# Autodesk Inventor assembly: McCrea_walle_drifter_walle
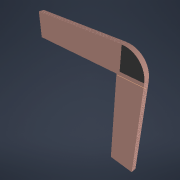
[picture p0: Inventor's stored thumbnail of the model, 180x180]
Saved by Autodesk Inventor 2022 (Build 260153000, 153)
## iProperties
Created: 2022-02-12
Part Number: McCrea_walle_drifter_walle
Document SubType Name: Assembly
Designer: MatusBarany
Author: MatusBarany
## Documents named in this file (4)
- C:\Users\MatusBarany\Documents\Inventor\wall-e\assembly\McCrea_walle_drifter_walle.iam
- C:\Users\MatusBarany\Documents\Inventor\wall-e\matus\plocha\McCrea_most_cesta_walle.ipt
- C:\Users\MatusBarany\Documents\Inventor\wall-e\matus\plocha\McCrea_zakruta_walle.ipt
- C:\Users\MatusBarany\Documents\Inventor\wall-e\assembly\McCrea_WALLE_bez_HEAD_walle.iam
## Components (6 placed, 3 different names)
1. McCrea_most_cesta_walle:1 — Mate:1, Flush:1, Mate:2, Mate:3, Flush:3, Mate:5, Mate:6
2. McCrea_zakruta_walle:1 — Mate:1, Flush:1, Mate:2, Mate:4, Flush:2
3. McCrea_WALLE_bez_HEAD_walle:1 [sub-assembly] — Mate:3
4. McCrea_most_cesta_walle:2 — Mate:4, Flush:2, Flush:3
5. McCrea_WALLE_bez_HEAD_walle:2 [sub-assembly] — Mate:5
6. McCrea_WALLE_bez_HEAD_walle:3 [sub-assembly] — Mate:6
## Relationships (9: Mate 6, Flush 3)
- Mate:1: McCrea_most_cesta_walle:1 ↔ McCrea_zakruta_walle:1
- Flush:1: McCrea_most_cesta_walle:1 ↔ McCrea_zakruta_walle:1
- Mate:2: McCrea_most_cesta_walle:1 ↔ McCrea_zakruta_walle:1
- Mate:3: McCrea_most_cesta_walle:1 ↔ McCrea_WALLE_bez_HEAD_walle:1
- Mate:4: McCrea_zakruta_walle:1 ↔ McCrea_most_cesta_walle:2
- Flush:2: McCrea_zakruta_walle:1 ↔ McCrea_most_cesta_walle:2
- Flush:3: McCrea_most_cesta_walle:1 ↔ McCrea_most_cesta_walle:2
- Mate:5: McCrea_most_cesta_walle:1 ↔ McCrea_WALLE_bez_HEAD_walle:2
- Mate:6: McCrea_most_cesta_walle:1 ↔ McCrea_WALLE_bez_HEAD_walle:3
